# Autodesk Inventor assembly: alltogether
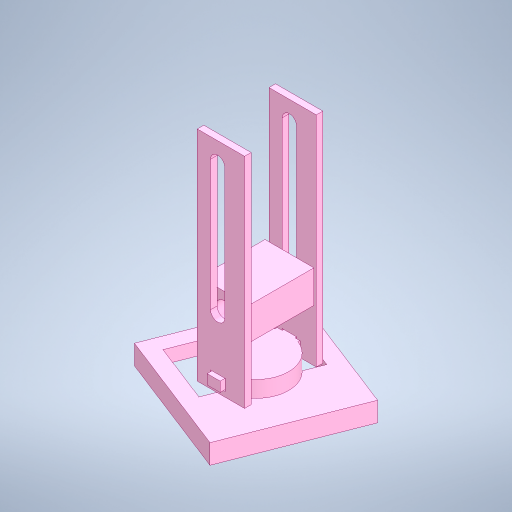
[picture p0: Inventor's stored thumbnail of the model, 512x512]
Saved by Autodesk Inventor 2024.3 (Build 283343000, 343)
## iProperties
Created: 2024-08-04
Part Number: alltogether
Document SubType Name: Assembly
Designer: compu
Author: compu
## Documents named in this file (5)
- C:\Users\compu\Documents\1Juan\1Facultad\9 Semestre\E1225 Taller de Sistemas Digitales\0Repository\BandTBS\Piezas\Partes 3D\soporte de camara\alltogether.iam
- C:\Users\compu\Documents\1Juan\1Facultad\9 Semestre\E1225 Taller de Sistemas Digitales\0Repository\BandTBS\Piezas\Partes 3D\soporte de camara\cam_socket.ipt
- C:\Users\compu\Documents\1Juan\1Facultad\9 Semestre\E1225 Taller de Sistemas Digitales\0Repository\BandTBS\Piezas\Partes 3D\soporte de camara\turntable.ipt
- C:\Users\compu\Documents\1Juan\1Facultad\9 Semestre\E1225 Taller de Sistemas Digitales\0Repository\BandTBS\Piezas\Partes 3D\soporte de camara\hammock_arms.ipt
- C:\Users\compu\Documents\1Juan\1Facultad\9 Semestre\E1225 Taller de Sistemas Digitales\0Repository\BandTBS\Piezas\Partes 3D\soporte de camara\stop_block.ipt
## Components (5 placed, 4 different names)
1. cam_socket:1 — Mate:1, Mate:2, Flush:1, Mate:5
2. turntable:1 — Mate:1, Mate:2, Flush:2, Mate:3, Mate:5, Mate:6, Mate:7, Mate:8, Mate:9, Mate:10, Mate:11
3. hammock_arms:1 — Mate:6, Mate:7, Mate:8, Mate:13, Mate:15
4. hammock_arms:2 — Mate:9, Mate:10, Mate:11, Mate:14
5. stop_block:1 — Mate:12, Mate:13, Mate:14, Mate:15
## Relationships (16: Mate 14, Flush 2)
- Mate:1: cam_socket:1 ↔ turntable:1
- Mate:2: cam_socket:1 ↔ turntable:1
- Flush:1: cam_socket:1
- Flush:2: turntable:1
- Mate:3: turntable:1
- Mate:5: cam_socket:1 ↔ turntable:1
- Mate:6: turntable:1 ↔ hammock_arms:1
- Mate:7: turntable:1 ↔ hammock_arms:1
- Mate:8: turntable:1 ↔ hammock_arms:1
- Mate:9: turntable:1 ↔ hammock_arms:2
- Mate:10: turntable:1 ↔ hammock_arms:2
- Mate:11: turntable:1 ↔ hammock_arms:2
- Mate:12: stop_block:1
- Mate:13: hammock_arms:1 ↔ stop_block:1
- Mate:14: hammock_arms:2 ↔ stop_block:1
- Mate:15: hammock_arms:1 ↔ stop_block:1
